# Autodesk Inventor assembly: assembly
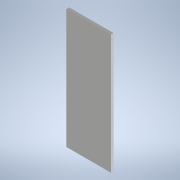
[picture p0: Inventor's stored thumbnail of the model, 180x180]
Saved by Autodesk Inventor 2020 (Build 240168000, 168)
## iProperties
Created: 2020-03-09
Part Number: assembly
Document SubType Name: Assembly
Designer: erwin
Author: erwin
## Documents named in this file (3)
- D:\GitHub\BeachMaid\platform-2\9mm_lid\assembly.iam
- D:\GitHub\BeachMaid\platform-2\9mm_lid\lid.ipt
- D:\GitHub\BeachMaid\platform-2\9mm_lid\middle.ipt
## Components (2 placed, 2 different names)
1. lid:1 — Flush:1
2. middle:1 — Flush:1
## Relationships (1: Flush 1)
- Flush:1: lid:1 ↔ middle:1
